# Autodesk Inventor assembly: Ensamble
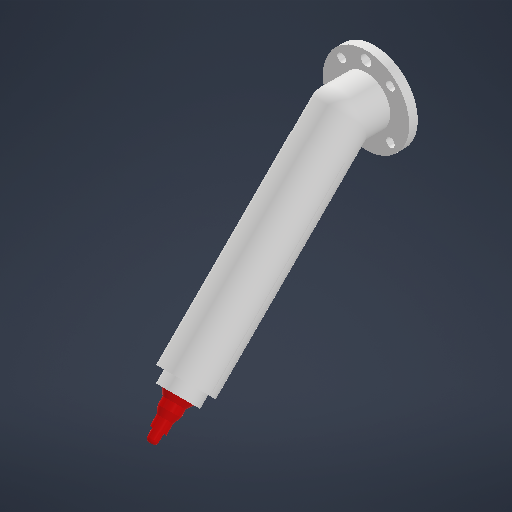
[picture p0: Inventor's stored thumbnail of the model, 512x512]
Saved by Autodesk Inventor 2026 (Build 300175000, 175)
## iProperties
Created: 2025-09-24
Part Number: Ensamble
Document SubType Name: Assembly
Designer: santi
Author: santi
## Documents named in this file (4)
- C:\Users\santi\Downloads\Ensamble v1\Ensamble.iam
- C:\Users\santi\Downloads\Ensamble v1\portam v1.ipt
- C:\Users\santi\Downloads\Ensamble v1\marcador v1.ipt
- C:\Users\santi\Downloads\Ensamble v1\shell v1.ipt
## Components (3 placed, 3 different names)
1. portam v1:1 — Mate:1, Flush:1, Flush:2, Mate:3, Flush:4, Mate:6, Mate:7, Mate:8, Mate:9, Mate:10
2. marcador v1:1 — Mate:2, Flush:3
3. shell v1:1 — Mate:6, Mate:7, Mate:8, Mate:9, Mate:10
## Relationships (14: Mate 10, Flush 4)
- Mate:1: portam v1:1
- Flush:1: portam v1:1
- Flush:2: portam v1:1
- Mate:2: marcador v1:1
- Mate:3: portam v1:1
- Mate:4
- Flush:3: marcador v1:1
- Flush:4: portam v1:1
- Mate:5
- Mate:6: portam v1:1 ↔ shell v1:1
- Mate:7: portam v1:1 ↔ shell v1:1
- Mate:8: portam v1:1 ↔ shell v1:1
- Mate:9: portam v1:1 ↔ shell v1:1
- Mate:10: portam v1:1 ↔ shell v1:1
